# Autodesk Inventor assembly: atras
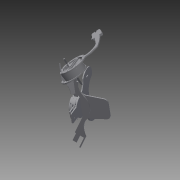
[picture p0: Inventor's stored thumbnail of the model, 180x180]
Saved by Autodesk Inventor 2015 (Build 190159000, 159)
## iProperties
Created: 2017-10-03
Part Number: atras
Document SubType Name: Assembly
Designer: macbook
Author: macbook
## Documents named in this file (12)
- C:\Users\Max\Dropbox\cosplay\atras.iam
- C:\Users\Max\Dropbox\cosplay\espalda\lados\brazo.ipt
- C:\Users\Max\Dropbox\cosplay\espalda\lados\base.ipt
- C:\Users\Max\Dropbox\cosplay\espalda\lados\medio.ipt
- C:\Users\Max\Dropbox\cosplay\espalda\lados\brazos.ipt
- C:\Users\Max\Dropbox\cosplay\espalda\base.ipt
- C:\Users\Max\Dropbox\cosplay\espalda\central.ipt
- C:\Users\Max\Dropbox\cosplay\espalda\centralmedio.ipt
- C:\Users\Max\Dropbox\cosplay\espalda\tapa.ipt
- C:\Users\Max\Dropbox\cosplay\espalda\lados\tapalarga.ipt
- C:\Users\Max\Dropbox\cosplay\espalda\lados\adelante.ipt
- C:\Users\Max\Dropbox\cosplay\espalda\lados\refuerzo.ipt
## Components (22 placed, 10 different names)
1. brazo:1 — Mate:1, Mate:2, Mate:3, Mate:5, Mate:6, Mate:10, Mate:11, Mate:12, Mate:26
2. base:1 — Mate:1, Mate:2, Mate:3, Mate:4, Mate:7, Mate:8, Mate:9, Mate:16, Mate:19
3. medio:1 — Rigid:2, Mate:5, Mate:6, Mate:17, Mate:18, Mate:20, Mate:21, Mate:22
4. medio:2 — Rigid:1, Rigid:3
5. medio:3 — Rigid:1, Rigid:2
6. medio:4 — Rigid:3, Rigid:4
7. medio:5 — Rigid:6, Mate:4
8. medio:6 — Rigid:5, Rigid:6
9. medio:7 — Rigid:4, Rigid:5
10. brazos:1 — Mate:7, Mate:8, Mate:9
11. brazos:2 — Mate:16, Mate:17, Mate:18
12. base:2 — Mate:10, Mate:11, Mate:12, Mate:13, Flush:1, Flush:2, Mate:27
13. central:1 — Rigid:7, Flush:1, Flush:2, Mate:14, Flush:3, Flush:4
14. central:2 — Rigid:7, Mate:13
15. centralmedio:1 — Mate:14, Flush:3, Flush:4, Mate:15, Flush:5, Flush:6
16. central:3 — Mate:15, Flush:5, Flush:6, Rigid:8
17. central:4 — Rigid:8, Rigid:9
18. tapa:1 — Rigid:9
19. brazos:3 — Mate:19, Mate:20, Mate:21, Mate:23, Mate:24
20. tapalarga:1 — Mate:22, Mate:23, Mate:24, Mate:25, Flush:7, Flush:8
21. adelante:1 — Mate:25, Flush:7, Flush:8
22. refuerzo:1 — Mate:26, Mate:27
## Relationships (44: Mate 27, WeldJoint 9, Flush 8)
- Mate:1: brazo:1 ↔ base:1
- Mate:2: brazo:1 ↔ base:1
- Mate:3: brazo:1 ↔ base:1
- Rigid:1 [WeldJoint]: medio:2 ↔ medio:3
- Rigid:2 [WeldJoint]: medio:1 ↔ medio:3
- Rigid:3 [WeldJoint]: medio:2 ↔ medio:4
- Rigid:4 [WeldJoint]: medio:4 ↔ medio:7
- Rigid:5 [WeldJoint]: medio:6 ↔ medio:7
- Rigid:6 [WeldJoint]: medio:5 ↔ medio:6
- Mate:4: base:1 ↔ medio:5
- Mate:5: brazo:1 ↔ medio:1
- Mate:6: brazo:1 ↔ medio:1
- Mate:7: base:1 ↔ brazos:1
- Mate:8: base:1 ↔ brazos:1
- Mate:9: base:1 ↔ brazos:1
- Mate:10: brazo:1 ↔ base:2
- Mate:11: brazo:1 ↔ base:2
- Mate:12: brazo:1 ↔ base:2
- Rigid:7 [WeldJoint]: central:1 ↔ central:2
- Mate:13: base:2 ↔ central:2
- Flush:1: base:2 ↔ central:1
- Flush:2: base:2 ↔ central:1
- Mate:14: central:1 ↔ centralmedio:1
- Flush:3: central:1 ↔ centralmedio:1
- Flush:4: central:1 ↔ centralmedio:1
- Mate:15: centralmedio:1 ↔ central:3
- Flush:5: centralmedio:1 ↔ central:3
- Flush:6: centralmedio:1 ↔ central:3
- Rigid:8 [WeldJoint]: central:3 ↔ central:4
- Rigid:9 [WeldJoint]: central:4 ↔ tapa:1
- Mate:16: base:1 ↔ brazos:2
- Mate:17: medio:1 ↔ brazos:2
- Mate:18: medio:1 ↔ brazos:2
- Mate:19: base:1 ↔ brazos:3
- Mate:20: medio:1 ↔ brazos:3
- Mate:21: medio:1 ↔ brazos:3
- Mate:22: medio:1 ↔ tapalarga:1
- Mate:23: brazos:3 ↔ tapalarga:1
- Mate:24: brazos:3 ↔ tapalarga:1
- Mate:25: tapalarga:1 ↔ adelante:1
- Flush:7: tapalarga:1 ↔ adelante:1
- Flush:8: tapalarga:1 ↔ adelante:1
- Mate:26: brazo:1 ↔ refuerzo:1
- Mate:27: base:2 ↔ refuerzo:1
